# Autodesk Inventor assembly: BoxBuild
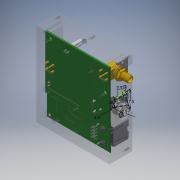
[picture p0: Inventor's stored thumbnail of the model, 180x180]
Saved by Autodesk Inventor 2019.4 (Build 234330000, 330)
## iProperties
Created: 2020-06-10
Part Number: BoxBuild
Document SubType Name: Assembly
Designer: ions
Author: ions
## Documents named in this file (8)
- Z:\Shared\Squareatron\BoxBuild.iam
- Z:\Shared\Squareatron\Box_V2.ipt
- Z:\Shared\Squareatron\squareatron.ipt
- Z:\Shared\Squareatron\DAC_Board_PCB.ipt
- Z:\Shared\Squareatron\DAC_GP.iam
- Z:\Shared\Squareatron\UCover_PWR.ipt
- Z:\Shared\Squareatron\UCover_SMA.ipt
- Z:\Shared\Squareatron\Lid.ipt
## Components (8 placed, 7 different names)
1. Box_V2:1 — Angle:1, Insert:1, Angle:2, Insert:5, Insert:6, Insert:7, Insert:8
2. squareatron:1 — Angle:1, Insert:1, Insert:2
3. DAC_Board_PCB:1 — Insert:2, Angle:2, Angle:3, Insert:3
4. DAC_GP:1 [sub-assembly] — Angle:3, Insert:3
5. UCover_PWR:1
6. UCover_SMA:1 — Insert:5
7. UCover_SMA:2 — Insert:6
8. Lid:1 — Insert:7, Insert:8
## Relationships (10: Insert 7, Angle 3)
- Angle:1 (270 deg): Box_V2:1 ↔ squareatron:1
- Insert:1 (-1.6 mm): Box_V2:1 ↔ squareatron:1
- Insert:2: squareatron:1 ↔ DAC_Board_PCB:1
- Angle:2 (0 deg): Box_V2:1 ↔ DAC_Board_PCB:1
- Angle:3 (180 deg): DAC_Board_PCB:1 ↔ DAC_GP:1
- Insert:3: DAC_Board_PCB:1 ↔ DAC_GP:1
- Insert:5 (-2 mm): Box_V2:1 ↔ UCover_SMA:1
- Insert:6 (-2 mm): Box_V2:1 ↔ UCover_SMA:2
- Insert:7 (-2 mm): Box_V2:1 ↔ Lid:1
- Insert:8 (-2 mm): Box_V2:1 ↔ Lid:1
